# Autodesk Inventor assembly: Oktokommander
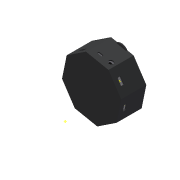
[picture p0: Inventor's stored thumbnail of the model, 180x180]
Saved by Autodesk Inventor 2018.2 (Build 222227000, 227)
## iProperties
Company: Fraunhofer ILT
Created: 2018-10-31
Part Number: Oktokommander
Material: geeigneten Werkstoff auswählen !
Document SubType Name: Assembly
Designer: N.Grubert
Title: =Description
Author: N.Grubert
## Documents named in this file (6)
- V:\A340\2018\DOKUMENTATION\COSIMA\COSIMA-Laserstar\CAD\Oktokommander\Oktokommander.iam
- V:\A340\2018\DOKUMENTATION\COSIMA\COSIMA-Laserstar\CAD\Oktagongehäuse\Oktagon.ipt
- V:\A340\2018\DOKUMENTATION\COSIMA\COSIMA-Laserstar\CAD\Oktagongehäuse\Oktagon_Deckel.ipt
- V:\A340\2018\DOKUMENTATION\COSIMA\COSIMA-Laserstar\CAD\Oktokommander\OktagonElektronik_Stage1.iam
- V:\A340\2018\DOKUMENTATION\COSIMA\COSIMA-Laserstar\CAD\Oktokommander\OktagonElektronik_Stage2.iam
- V:\A340\2018\DOKUMENTATION\COSIMA\COSIMA-Laserstar\CAD\Oktokommander\OktagonElektronik_Stage3.iam
## Components (5 placed, 5 different names)
1. Oktagon:1 — Passend:2, Passend:3, Passend:5, Passend:6, Passend:9, Passend:13, Passend:18, Passend:19, Passend:20, Passend:21, Fluchtend:1, Fluchtend:2
2. Oktagon_Deckel:1 — Passend:9, Fluchtend:1, Fluchtend:2
3. OktagonElektronik_Stage1:1 [sub-assembly] — Passend:2, Passend:3, Passend:18
4. OktagonElektronik_Stage2:1 [sub-assembly] — Passend:5, Passend:6, Passend:13
5. OktagonElektronik_Stage3:1 [sub-assembly] — Passend:19, Passend:20, Passend:21
## Relationships (12: Mate 10, Flush 2)
- Passend:2 [Mate] (3.5 mm): Oktagon:1 ↔ OktagonElektronik_Stage1:1
- Passend:3 [Mate] (3.5 mm): Oktagon:1 ↔ OktagonElektronik_Stage1:1
- Passend:5 [Mate] (0.5 mm): Oktagon:1 ↔ OktagonElektronik_Stage2:1
- Passend:6 [Mate] (0.5 mm): Oktagon:1 ↔ OktagonElektronik_Stage2:1
- Passend:9 [Mate]: Oktagon:1 ↔ Oktagon_Deckel:1
- Passend:13 [Mate]: Oktagon:1 ↔ OktagonElektronik_Stage2:1
- Passend:18 [Mate]: Oktagon:1 ↔ OktagonElektronik_Stage1:1
- Passend:19 [Mate]: Oktagon:1 ↔ OktagonElektronik_Stage3:1
- Passend:20 [Mate] (0.5 mm): Oktagon:1 ↔ OktagonElektronik_Stage3:1
- Passend:21 [Mate] (0.5 mm): Oktagon:1 ↔ OktagonElektronik_Stage3:1
- Fluchtend:1 [Flush]: Oktagon:1 ↔ Oktagon_Deckel:1
- Fluchtend:2 [Flush]: Oktagon:1 ↔ Oktagon_Deckel:1
